# Autodesk Inventor assembly: КВ33.044.900 - Каретка оси X
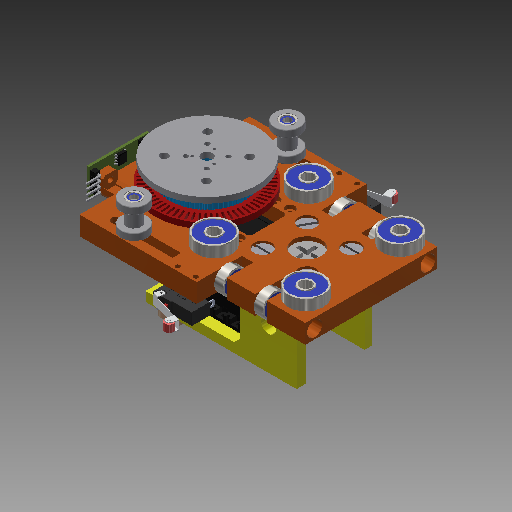
[picture p0: Inventor's stored thumbnail of the model, 512x512]
Saved by Autodesk Inventor 2019 (Build 230136000, 136)
## iProperties
Created: 2019-08-08
Part Number: КВ33.044.900 - Каретка оси X
Material: Типовые
Document SubType Name: Assembly
Designer: user
Author: user
## Documents named in this file (16)
- E:\IVAN\Kvantoriada2019\optimal_gripper\hardware\КВ33.044.400 - Каретка оси X.iam
- E:\IVAN\Kvantoriada2019\optimal_gripper\hardware\КВ33.044.401 - Щека каретки X.ipt
- E:\IVAN\Kvantoriada2019\optimal_gripper\hardware\Стандартные изделия\Подшипник 624Z.ipt
- E:\IVAN\Kvantoriada2019\optimal_gripper\hardware\Стандартные изделия\Подшипник 626Z.ipt
- E:\IVAN\Kvantoriada2019\optimal_gripper\hardware\Стандартные изделия\Винт М8х25 с потайной головкой.ipt
- E:\IVAN\Kvantoriada2019\optimal_gripper\hardware\Стандартные изделия\Винт М5х10 с потайной головкой.ipt
- E:\IVAN\Kvantoriada2019\optimal_gripper\hardware\Стандартные изделия\Сервомотор Dynamixel AX-12A\AX-12.iam
- E:\IVAN\Kvantoriada2019\optimal_gripper\hardware\Стандартные изделия\Проставка 6.5 мм.ipt
- E:\IVAN\Kvantoriada2019\optimal_gripper\hardware\Стандартные изделия\Колесо оптического датчика.ipt
- E:\IVAN\Kvantoriada2019\optimal_gripper\hardware\Стандартные изделия\Шкив большой Makeblock.ipt
- E:\IVAN\Kvantoriada2019\optimal_gripper\hardware\Стандартные изделия\Боковина шкива.ipt
- E:\IVAN\Kvantoriada2019\optimal_gripper\hardware\Стандартные изделия\Датчик оптический стандартный.ipt
- E:\IVAN\Kvantoriada2019\optimal_gripper\hardware\Стандартные изделия\Концевик механический.ipt
- E:\IVAN\Kvantoriada2019\optimal_gripper\hardware\Стандартные изделия\Шкив плоский Makeblock сборка.iam
- E:\IVAN\Kvantoriada2019\optimal_gripper\hardware\КВ33.044.405 - Крепеж ремня оси Y.ipt
- E:\IVAN\Kvantoriada2019\optimal_gripper\hardware\КВ33.044.406 - Прижим ремня.ipt
## Components (26 placed, 15 different names)
1. КВ33.044.401 - Щека каретки X:1 — Совмещение:1, Совмещение:2, Совмещение:3, Совмещение:4, Совмещение:5, Совмещение:6, Совмещение:7, Совмещение:8, Совмещение:9, Совмещение:10, Совмещение:11, Совмещение:12, Совмещение:13, Совмещение:14, Совмещение:15, Совмещение:16, Совмещение:17, Заподлицо:1, Совмещение:18, Заподлицо:2, Совмещение:19, Заподлицо:3, Совмещение:20, Заподлицо:4, Совмещение:21, Заподлицо:5, Совмещение:39, Совмещение:40, Заподлицо:6, Совмещение:41, Совмещение:42, Совмещение:43, Совмещение:44, Совмещение:45, Совмещение:46, Касательность:1, Касательность:2, Совмещение:47, Совмещение:48, Совмещение:53, Совмещение:54, Совмещение:55
2. Подшипник 624Z:1 — Совмещение:1, Совмещение:2
3. Подшипник 624Z:2 — Совмещение:3, Совмещение:4
4. Подшипник 624Z:3 — Совмещение:7, Совмещение:8
5. Подшипник 624Z:4 — Совмещение:5, Совмещение:6
6. Подшипник 626Z:1 — Совмещение:9, Совмещение:10
7. Подшипник 626Z:2 — Совмещение:13, Совмещение:14
8. Подшипник 626Z:3 — Совмещение:11, Совмещение:12
9. Подшипник 626Z:4 — Совмещение:15, Совмещение:16
10. Винт М8х25 с потайной головкой:1 — Совмещение:17, Заподлицо:1
11. Винт М5х10 с потайной головкой:1 — Совмещение:19, Заподлицо:3
12. Винт М5х10 с потайной головкой:2 — Совмещение:21, Заподлицо:5
13. Винт М5х10 с потайной головкой:3 — Совмещение:18, Заподлицо:2
14. Винт М5х10 с потайной головкой:4 — Совмещение:20, Заподлицо:4
15. AX-12:1 [sub-assembly] — Совмещение:53, Совмещение:54, Совмещение:55, Совмещение:56, Совмещение:57, Совмещение:58, Совмещение:59, Совмещение:60
16. Проставка 6.5 мм:1 — Совмещение:27, Совмещение:28, Совмещение:29, Совмещение:59, Совмещение:60
17. Колесо оптического датчика:1 — Совмещение:27, Совмещение:28, Совмещение:29, Совмещение:30, Совмещение:31, Совмещение:32
18. Шкив большой Makeblock:1 — Совмещение:30, Совмещение:31, Совмещение:32, Совмещение:33, Совмещение:34, Совмещение:35
19. Боковина шкива:1 — Совмещение:33, Совмещение:34, Совмещение:35
20. Датчик оптический стандартный:1 — Совмещение:39, Совмещение:40, Заподлицо:6
21. Концевик механический:1 — Совмещение:41, Совмещение:42, Совмещение:43
22. Концевик механический:2 — Совмещение:44, Совмещение:45, Совмещение:46
23. Шкив плоский Makeblock сборка:1 [sub-assembly] — Касательность:1, Совмещение:48
24. Шкив плоский Makeblock сборка:2 [sub-assembly] — Касательность:2, Совмещение:47
25. КВ33.044.405 - Крепеж ремня оси Y:1 — Совмещение:52, Касательность:3, Касательность:4, Совмещение:56, Совмещение:57, Совмещение:58
26. КВ33.044.406 - Прижим ремня:1 — Совмещение:52, Касательность:3, Касательность:4
## Relationships (59: Mate 49, Flush 6, Tangent 4)
- Совмещение:1 [Mate]: КВ33.044.401 - Щека каретки X:1 ↔ Подшипник 624Z:1
- Совмещение:2 [Mate] (0.5 mm): КВ33.044.401 - Щека каретки X:1 ↔ Подшипник 624Z:1
- Совмещение:3 [Mate]: КВ33.044.401 - Щека каретки X:1 ↔ Подшипник 624Z:2
- Совмещение:4 [Mate] (0.5 mm): КВ33.044.401 - Щека каретки X:1 ↔ Подшипник 624Z:2
- Совмещение:5 [Mate] (0.5 mm): КВ33.044.401 - Щека каретки X:1 ↔ Подшипник 624Z:4
- Совмещение:6 [Mate]: КВ33.044.401 - Щека каретки X:1 ↔ Подшипник 624Z:4
- Совмещение:7 [Mate]: КВ33.044.401 - Щека каретки X:1 ↔ Подшипник 624Z:3
- Совмещение:8 [Mate] (0.5 mm): КВ33.044.401 - Щека каретки X:1 ↔ Подшипник 624Z:3
- Совмещение:9 [Mate]: КВ33.044.401 - Щека каретки X:1 ↔ Подшипник 626Z:1
- Совмещение:10 [Mate] (2 mm): КВ33.044.401 - Щека каретки X:1 ↔ Подшипник 626Z:1
- Совмещение:11 [Mate]: КВ33.044.401 - Щека каретки X:1 ↔ Подшипник 626Z:3
- Совмещение:12 [Mate] (2 mm): КВ33.044.401 - Щека каретки X:1 ↔ Подшипник 626Z:3
- Совмещение:13 [Mate]: КВ33.044.401 - Щека каретки X:1 ↔ Подшипник 626Z:2
- Совмещение:14 [Mate] (2 mm): КВ33.044.401 - Щека каретки X:1 ↔ Подшипник 626Z:2
- Совмещение:15 [Mate]: КВ33.044.401 - Щека каретки X:1 ↔ Подшипник 626Z:4
- Совмещение:16 [Mate] (2 mm): КВ33.044.401 - Щека каретки X:1 ↔ Подшипник 626Z:4
- Совмещение:17 [Mate]: КВ33.044.401 - Щека каретки X:1 ↔ Винт М8х25 с потайной головкой:1
- Заподлицо:1 [Flush] (2 mm): КВ33.044.401 - Щека каретки X:1 ↔ Винт М8х25 с потайной головкой:1
- Совмещение:18 [Mate]: КВ33.044.401 - Щека каретки X:1 ↔ Винт М5х10 с потайной головкой:3
- Заподлицо:2 [Flush] (1 mm): КВ33.044.401 - Щека каретки X:1 ↔ Винт М5х10 с потайной головкой:3
- Совмещение:19 [Mate]: КВ33.044.401 - Щека каретки X:1 ↔ Винт М5х10 с потайной головкой:1
- Заподлицо:3 [Flush] (1 mm): КВ33.044.401 - Щека каретки X:1 ↔ Винт М5х10 с потайной головкой:1
- Совмещение:20 [Mate]: КВ33.044.401 - Щека каретки X:1 ↔ Винт М5х10 с потайной головкой:4
- Заподлицо:4 [Flush] (1 mm): КВ33.044.401 - Щека каретки X:1 ↔ Винт М5х10 с потайной головкой:4
- Совмещение:21 [Mate]: КВ33.044.401 - Щека каретки X:1 ↔ Винт М5х10 с потайной головкой:2
- Заподлицо:5 [Flush] (1 mm): КВ33.044.401 - Щека каретки X:1 ↔ Винт М5х10 с потайной головкой:2
- Совмещение:27 [Mate]: Проставка 6.5 мм:1 ↔ Колесо оптического датчика:1
- Совмещение:28 [Mate]: Проставка 6.5 мм:1 ↔ Колесо оптического датчика:1
- Совмещение:29 [Mate]: Проставка 6.5 мм:1 ↔ Колесо оптического датчика:1
- Совмещение:30 [Mate]: Колесо оптического датчика:1 ↔ Шкив большой Makeblock:1
- Совмещение:31 [Mate]: Колесо оптического датчика:1 ↔ Шкив большой Makeblock:1
- Совмещение:32 [Mate]: Колесо оптического датчика:1 ↔ Шкив большой Makeblock:1
- Совмещение:33 [Mate]: Шкив большой Makeblock:1 ↔ Боковина шкива:1
- Совмещение:34 [Mate]: Шкив большой Makeblock:1 ↔ Боковина шкива:1
- Совмещение:35 [Mate]: Шкив большой Makeblock:1 ↔ Боковина шкива:1
- Совмещение:39 [Mate] (10 mm): КВ33.044.401 - Щека каретки X:1 ↔ Датчик оптический стандартный:1
- Совмещение:40 [Mate] (-4.7 mm): КВ33.044.401 - Щека каретки X:1 ↔ Датчик оптический стандартный:1
- Заподлицо:6 [Flush] (15 mm): КВ33.044.401 - Щека каретки X:1 ↔ Датчик оптический стандартный:1
- Совмещение:41 [Mate]: КВ33.044.401 - Щека каретки X:1 ↔ Концевик механический:1
- Совмещение:42 [Mate]: КВ33.044.401 - Щека каретки X:1 ↔ Концевик механический:1
- Совмещение:43 [Mate]: КВ33.044.401 - Щека каретки X:1 ↔ Концевик механический:1
- Совмещение:44 [Mate]: КВ33.044.401 - Щека каретки X:1 ↔ Концевик механический:2
- Совмещение:45 [Mate]: КВ33.044.401 - Щека каретки X:1 ↔ Концевик механический:2
- Совмещение:46 [Mate]: КВ33.044.401 - Щека каретки X:1 ↔ Концевик механический:2
- Касательность:1 [Tangent]: КВ33.044.401 - Щека каретки X:1 ↔ Шкив плоский Makeblock сборка:1
- Касательность:2 [Tangent]: КВ33.044.401 - Щека каретки X:1 ↔ Шкив плоский Makeblock сборка:2
- Совмещение:47 [Mate]: КВ33.044.401 - Щека каретки X:1 ↔ Шкив плоский Makeblock сборка:2
- Совмещение:48 [Mate]: КВ33.044.401 - Щека каретки X:1 ↔ Шкив плоский Makeblock сборка:1
- Совмещение:52 [Mate]: КВ33.044.405 - Крепеж ремня оси Y:1 ↔ КВ33.044.406 - Прижим ремня:1
- Касательность:3 [Tangent]: КВ33.044.405 - Крепеж ремня оси Y:1 ↔ КВ33.044.406 - Прижим ремня:1
- Касательность:4 [Tangent]: КВ33.044.405 - Крепеж ремня оси Y:1 ↔ КВ33.044.406 - Прижим ремня:1
- Совмещение:53 [Mate]: КВ33.044.401 - Щека каретки X:1 ↔ AX-12:1
- Совмещение:54 [Mate]: КВ33.044.401 - Щека каретки X:1 ↔ AX-12:1
- Совмещение:55 [Mate]: КВ33.044.401 - Щека каретки X:1 ↔ AX-12:1
- Совмещение:56 [Mate]: AX-12:1 ↔ КВ33.044.405 - Крепеж ремня оси Y:1
- Совмещение:57 [Mate]: AX-12:1 ↔ КВ33.044.405 - Крепеж ремня оси Y:1
- Совмещение:58 [Mate]: AX-12:1 ↔ КВ33.044.405 - Крепеж ремня оси Y:1
- Совмещение:59 [Mate]: AX-12:1 ↔ Проставка 6.5 мм:1
- Совмещение:60 [Mate]: AX-12:1 ↔ Проставка 6.5 мм:1
